# Autodesk Inventor assembly: КВ33.044.300 -  Сборка мотора Makeblock с крепление
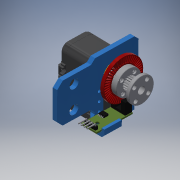
[picture p0: Inventor's stored thumbnail of the model, 180x180]
Saved by Autodesk Inventor 2019 (Build 230136000, 136)
## iProperties
Created: 2019-07-17
Part Number: КВ33.044.300 -  Сборка мотора Makeblock с крепление
Material: Типовые
Document SubType Name: Assembly
Designer: Петров Иван
Author: Петров Иван
## Documents named in this file (7)
- C:\Users\user\Documents\Kvantoriada2019\optimal_gripper\hardware\КВ33.044.300 -  Сборка сервомотора Makeblock с крепление.iam
- C:\Users\user\Documents\Kvantoriada2019\optimal_gripper\hardware\КВ33.044.301 - Деражатель мотора.ipt
- C:\Users\user\Documents\Kvantoriada2019\optimal_gripper\hardware\проставка.ipt
- C:\Users\user\Documents\Kvantoriada2019\optimal_gripper\hardware\колесо.ipt
- C:\Users\user\Documents\Kvantoriada2019\optimal_gripper\hardware\шкив.ipt
- C:\Users\user\Documents\Kvantoriada2019\optimal_gripper\hardware\Стандартные изделия\Сервомотор Dynamixel AX-12A\ax-12a.iam
- C:\Users\user\Documents\Kvantoriada2019\optimal_gripper\hardware\Стандартные изделия\Оптический датчик.ipt
## Components (6 placed, 6 different names)
1. КВ33.044.301 - Деражатель мотора:1 — Совмещение:1, Совмещение:2, Совмещение:7, Совмещение:8, Совмещение:9, Заподлицо:1, Заподлицо:2, Совмещение:10
2. проставка:1 — Совмещение:1, Совмещение:2, Совмещение:3, Совмещение:4
3. колесо:1 — Совмещение:3, Совмещение:4, Совмещение:5, Совмещение:6
4. шкив:1 — Совмещение:5, Совмещение:6
5. Оптический датчик:1 — Заподлицо:1, Заподлицо:2, Совмещение:10
6. ax-12a:1 [sub-assembly] — Совмещение:7, Совмещение:8, Совмещение:9
## Relationships (12: Mate 10, Flush 2)
- Совмещение:1 [Mate]: КВ33.044.301 - Деражатель мотора:1 ↔ проставка:1
- Совмещение:2 [Mate]: КВ33.044.301 - Деражатель мотора:1 ↔ проставка:1
- Совмещение:3 [Mate]: проставка:1 ↔ колесо:1
- Совмещение:4 [Mate]: проставка:1 ↔ колесо:1
- Совмещение:5 [Mate]: колесо:1 ↔ шкив:1
- Совмещение:6 [Mate]: колесо:1 ↔ шкив:1
- Совмещение:7 [Mate]: КВ33.044.301 - Деражатель мотора:1 ↔ ax-12a:1
- Совмещение:8 [Mate]: КВ33.044.301 - Деражатель мотора:1 ↔ ax-12a:1
- Совмещение:9 [Mate]: КВ33.044.301 - Деражатель мотора:1 ↔ ax-12a:1
- Заподлицо:1 [Flush] (11 mm): КВ33.044.301 - Деражатель мотора:1 ↔ Оптический датчик:1
- Заподлицо:2 [Flush] (15 mm): КВ33.044.301 - Деражатель мотора:1 ↔ Оптический датчик:1
- Совмещение:10 [Mate]: КВ33.044.301 - Деражатель мотора:1 ↔ Оптический датчик:1
